# Autodesk Inventor assembly: climber
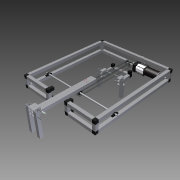
[picture p0: Inventor's stored thumbnail of the model, 180x180]
Saved by Autodesk Inventor 2011 (Build 150239000, 239)
## iProperties
Created: 2013-01-19
Part Number: climber
Document SubType Name: Assembly
Designer: Danny
Author: Danny
## Documents named in this file (18)
- C:\Users\Danny\Documents\GitHub\2013CAD\2013 robot\Spiderbot\climber.iam
- C:\Users\Danny\Documents\GitHub\2013CAD\2013 robot\Spiderbot\28 in 1-16.ipt
- C:\Users\Danny\Documents\GitHub\2013CAD\2013 robot\Spiderbot\24 in 1-16.ipt
- C:\Users\Danny\Documents\GitHub\2013CAD\2013 robot\Spiderbot\2 in 1-16.ipt
- C:\Users\Danny\Documents\GitHub\2013CAD\COTS parts\Plastic_Tubing_Connectors\3-way corner.ipt
- C:\Users\Danny\Documents\GitHub\2013CAD\2013 robot\Spiderbot\cim motor.ipt
- C:\Users\Danny\Documents\GitHub\2013CAD\2013 robot\Spiderbot\cim p80 gearbox.ipt
- C:\Users\Danny\Documents\GitHub\2013CAD\2013 robot\Spiderbot\sprocket.ipt
- C:\Users\Danny\Documents\GitHub\2013CAD\2013 robot\Spiderbot\axle bearing.ipt
- C:\Users\Danny\Documents\GitHub\2013CAD\2013 robot\Spiderbot\30 in 1-2 axle.ipt
- C:\Users\Danny\Documents\GitHub\2013CAD\2013 robot\Spiderbot\climber\Design Accelerator\Key Connection1.iam
- C:\Users\Danny\Documents\GitHub\2013CAD\2013 robot\Spiderbot\chainparts.ipt
- C:\Users\Danny\Documents\GitHub\2013CAD\2013 robot\Spiderbot\screwpin idk man.ipt
- C:\Users\Danny\Documents\GitHub\2013CAD\2013 robot\Spiderbot\short hex bolt.ipt
- C:\Users\Danny\Documents\GitHub\2013CAD\2013 robot\Spiderbot\nylock nut.ipt
- C:\Users\Danny\Documents\GitHub\2013CAD\2013 robot\Spiderbot\longarms.iam
- C:\Users\Danny\Documents\GitHub\2013CAD\2013 robot\Spiderbot\8 in 1-16.ipt
- C:\Users\Danny\Documents\GitHub\2013CAD\2013 robot\Spiderbot\longlongerarms.iam
## Components (55 placed, 17 different names)
1. 28 in 1-16:1 — Mate:26, Flush:57, Flush:58, Flush:59, Flush:60
2. 28 in 1-16:2 — Mate:1, Flush:1, Flush:2, Flush:3, Mate:5, Flush:9, Flush:10, Mate:56, Flush:75
3. 28 in 1-16:3 — Mate:4, Flush:7, Flush:8, Mate:6, Flush:11, Flush:12, Mate:57, Flush:76, Flush:77
4. 28 in 1-16:4 — Mate:25, Flush:53, Flush:54, Flush:55, Flush:56
5. 24 in 1-16:1 — Mate:27, Flush:61, Flush:62, Flush:63, Flush:64, Mate:72, Flush:78, Mate:73
6. 24 in 1-16:2 — Mate:2, Flush:3, Flush:4, Mate:3, Flush:5, Flush:6, Mate:65, Mate:70, Mate:71
7. 2 in 1-16:1 — Mate:14, Flush:27, Flush:28, Mate:19, Flush:37, Flush:38
8. 2 in 1-16:2 — Mate:13, Flush:25, Flush:26, Mate:20, Flush:39, Flush:40
9. 2 in 1-16:3 — Mate:11, Flush:21, Flush:22, Mate:21, Flush:41, Flush:42
10. 2 in 1-16:4 — Mate:12, Flush:23, Flush:24, Mate:22, Flush:43, Flush:44
11. 3-way corner:1 — Mate:5, Flush:9, Flush:10, Mate:14, Flush:27, Flush:28, Mate:79, Flush:82, Flush:83
12. 3-way corner:2 — Mate:1, Flush:1, Flush:2, Mate:2, Flush:4, Mate:15, Flush:29, Flush:30
13. 3-way corner:3 — Mate:11, Flush:21, Flush:22, Flush:84
14. 3-way corner:4 — Mate:12, Flush:23, Flush:24, Mate:82, Flush:89, Flush:91
15. 3-way corner:5 — Mate:19, Flush:37, Flush:38, Mate:26, Flush:57, Flush:58, Mate:77, Flush:80, Flush:81
16. 3-way corner:6 — Mate:18, Flush:35, Flush:36, Flush:55, Flush:56, Flush:63, Flush:64
17. 3-way corner:7 — Mate:22, Flush:43, Flush:44, Mate:80, Flush:85, Flush:86
18. 3-way corner:8 — Mate:6, Flush:11, Flush:12, Mate:13, Flush:25, Flush:26, Flush:90
19. 3-way corner:9 — Mate:3, Flush:5, Flush:6, Mate:4, Flush:7, Flush:8, Mate:16, Flush:31, Flush:32
20. 3-way corner:10 — Mate:17, Flush:33, Flush:34, Flush:59, Flush:60, Mate:27, Flush:61, Flush:62
21. 2 in 1-16:5 — Mate:15, Flush:29, Flush:30, Mate:17, Flush:33, Flush:34
22. 2 in 1-16:6 — Mate:16, Flush:31, Flush:32, Mate:18, Flush:35, Flush:36
23. 3-way corner:11 — Mate:20, Flush:39, Flush:40, Mate:25, Flush:53, Flush:54, Mate:81, Flush:87, Flush:88
24. 3-way corner:12 — Mate:21, Flush:41, Flush:42, Mate:78
25. cim motor:1 — Mate:48
26. cim p80 gearbox:1 — Mate:32, Mate:34, Flush:69, Mate:48, Mate:65
27. sprocket:2 — Mate:32, Flush:69, Mate:67
28. sprocket:3 — Mate:34, Mate:69
29. Key Connection:1 [sub-assembly] — Mate:63, Mate:64
30. 30 in 1-2 axle:2 — Mate:58, Mate:59, Flush:77, Mate:60, Mate:61, Mate:62, Mate:63, Mate:64
31. axle bearing:3 — Mate:57, Flush:76, Mate:59
32. axle bearing:4 — Mate:56, Flush:75, Mate:58
33. sprocket:7 — Mate:60, Mate:68
34. sprocket:8 — Mate:61, Mate:62, Mate:66
35. chainparts:1 — Mate:68, Mate:69, Mate:88, Mate:89
36. chainparts:2 — Mate:66, Mate:67, Mate:76, Flush:79, Mate:87, Mate:90, Mate:91
37. screwpin idk man:1
38. screwpin idk man:2 — Mate:70, Mate:71
39. 2 in 1-16:7 — Mate:72, Flush:78, Mate:75
40. Chassis_HexBolt_375x16x7_AndyMark_am-1055:2 — Mate:73, Mate:74
41. nylock nut:1 — Mate:74, Mate:75
42. longarms:1 [sub-assembly] — Mate:76, Flush:79, Mate:83, Mate:84, Mate:85, Mate:86
43. 8 in 1-16:1 — Mate:80, Flush:85, Flush:86, Mate:81, Flush:87, Flush:88
44. 8 in 1-16:2 — Mate:79, Flush:82, Flush:83, Flush:84
45. 8 in 1-16:3 — Mate:77, Flush:80, Flush:81, Mate:78
46. 8 in 1-16:4 — Mate:82, Flush:89, Flush:90, Flush:91
47. screwpin idk man:3 — Mate:83
48. screwpin idk man:4 — Mate:84
49. screwpin idk man:5 — Mate:85
50. screwpin idk man:6 — Mate:86
51. longlongerarms:1 [sub-assembly] — Mate:87
52. screwpin idk man:7 — Mate:89
53. screwpin idk man:8 — Mate:91
54. screwpin idk man:9 — Mate:88
55. screwpin idk man:10 — Mate:90
## Relationships (126: Flush 66, Mate 60)
- Mate:1: 28 in 1-16:2 ↔ 3-way corner:2
- Flush:1: 28 in 1-16:2 ↔ 3-way corner:2
- Flush:2: 28 in 1-16:2 ↔ 3-way corner:2
- Mate:2: 24 in 1-16:2 ↔ 3-way corner:2
- Flush:3: 28 in 1-16:2 ↔ 24 in 1-16:2
- Flush:4: 24 in 1-16:2 ↔ 3-way corner:2
- Mate:3: 24 in 1-16:2 ↔ 3-way corner:9
- Flush:5: 24 in 1-16:2 ↔ 3-way corner:9
- Flush:6: 24 in 1-16:2 ↔ 3-way corner:9
- Mate:4: 28 in 1-16:3 ↔ 3-way corner:9
- Flush:7: 28 in 1-16:3 ↔ 3-way corner:9
- Flush:8: 28 in 1-16:3 ↔ 3-way corner:9
- Mate:5: 28 in 1-16:2 ↔ 3-way corner:1
- Flush:9: 28 in 1-16:2 ↔ 3-way corner:1
- Flush:10: 28 in 1-16:2 ↔ 3-way corner:1
- Mate:6: 28 in 1-16:3 ↔ 3-way corner:8
- Flush:11: 28 in 1-16:3 ↔ 3-way corner:8
- Flush:12: 28 in 1-16:3 ↔ 3-way corner:8
- Mate:11: 2 in 1-16:3 ↔ 3-way corner:3
- Flush:21: 2 in 1-16:3 ↔ 3-way corner:3
- Flush:22: 2 in 1-16:3 ↔ 3-way corner:3
- Mate:12: 2 in 1-16:4 ↔ 3-way corner:4
- Flush:23: 2 in 1-16:4 ↔ 3-way corner:4
- Flush:24: 2 in 1-16:4 ↔ 3-way corner:4
- Mate:13: 2 in 1-16:2 ↔ 3-way corner:8
- Flush:25: 2 in 1-16:2 ↔ 3-way corner:8
- Flush:26: 2 in 1-16:2 ↔ 3-way corner:8
- Mate:14: 2 in 1-16:1 ↔ 3-way corner:1
- Flush:27: 2 in 1-16:1 ↔ 3-way corner:1
- Flush:28: 2 in 1-16:1 ↔ 3-way corner:1
- Mate:15: 3-way corner:2 ↔ 2 in 1-16:5
- Flush:29: 3-way corner:2 ↔ 2 in 1-16:5
- Flush:30: 3-way corner:2 ↔ 2 in 1-16:5
- Mate:16: 3-way corner:9 ↔ 2 in 1-16:6
- Flush:31: 3-way corner:9 ↔ 2 in 1-16:6
- Flush:32: 3-way corner:9 ↔ 2 in 1-16:6
- Mate:17: 3-way corner:10 ↔ 2 in 1-16:5
- Flush:33: 3-way corner:10 ↔ 2 in 1-16:5
- Flush:34: 3-way corner:10 ↔ 2 in 1-16:5
- Mate:18: 3-way corner:6 ↔ 2 in 1-16:6
- Flush:35: 3-way corner:6 ↔ 2 in 1-16:6
- Flush:36: 3-way corner:6 ↔ 2 in 1-16:6
- Mate:19: 2 in 1-16:1 ↔ 3-way corner:5
- Flush:37: 2 in 1-16:1 ↔ 3-way corner:5
- Flush:38: 2 in 1-16:1 ↔ 3-way corner:5
- Mate:20: 2 in 1-16:2 ↔ 3-way corner:11
- Flush:39: 2 in 1-16:2 ↔ 3-way corner:11
- Flush:40: 2 in 1-16:2 ↔ 3-way corner:11
- Mate:21: 2 in 1-16:3 ↔ 3-way corner:12
- Flush:41: 2 in 1-16:3 ↔ 3-way corner:12
- Flush:42: 2 in 1-16:3 ↔ 3-way corner:12
- Mate:22: 2 in 1-16:4 ↔ 3-way corner:7
- Flush:43: 2 in 1-16:4 ↔ 3-way corner:7
- Flush:44: 2 in 1-16:4 ↔ 3-way corner:7
- Mate:25: 28 in 1-16:4 ↔ 3-way corner:11
- Flush:53: 28 in 1-16:4 ↔ 3-way corner:11
- Flush:54: 28 in 1-16:4 ↔ 3-way corner:11
- Flush:55: 28 in 1-16:4 ↔ 3-way corner:6
- Flush:56: 28 in 1-16:4 ↔ 3-way corner:6
- Mate:26: 28 in 1-16:1 ↔ 3-way corner:5
- Flush:57: 28 in 1-16:1 ↔ 3-way corner:5
- Flush:58: 28 in 1-16:1 ↔ 3-way corner:5
- Flush:59: 28 in 1-16:1 ↔ 3-way corner:10
- Flush:60: 28 in 1-16:1 ↔ 3-way corner:10
- Mate:27: 24 in 1-16:1 ↔ 3-way corner:10
- Flush:61: 24 in 1-16:1 ↔ 3-way corner:10
- Flush:62: 24 in 1-16:1 ↔ 3-way corner:10
- Flush:63: 24 in 1-16:1 ↔ 3-way corner:6
- Flush:64: 24 in 1-16:1 ↔ 3-way corner:6
- Mate:32: cim p80 gearbox:1 ↔ sprocket:2
- Mate:34: cim p80 gearbox:1 ↔ sprocket:3
- Flush:69: cim p80 gearbox:1 ↔ sprocket:2
- Mate:48: cim motor:1 ↔ cim p80 gearbox:1
- Mate:56: 28 in 1-16:2 ↔ axle bearing:4
- Flush:75: 28 in 1-16:2 ↔ axle bearing:4
- Mate:57: 28 in 1-16:3 ↔ axle bearing:3
- Flush:76: 28 in 1-16:3 ↔ axle bearing:3
- Mate:58: 30 in 1-2 axle:2 ↔ axle bearing:4
- Mate:59: 30 in 1-2 axle:2 ↔ axle bearing:3
- Flush:77: 28 in 1-16:3 ↔ 30 in 1-2 axle:2
- Mate:60: 30 in 1-2 axle:2 ↔ sprocket:7
- Mate:61: 30 in 1-2 axle:2 ↔ sprocket:8
- Mate:62: 30 in 1-2 axle:2 ↔ sprocket:8
- Mate:63: Key Connection:1 ↔ 30 in 1-2 axle:2
- Mate:64: Key Connection:1 ↔ 30 in 1-2 axle:2
- Mate:65: 24 in 1-16:2 ↔ cim p80 gearbox:1
- Mate:66: sprocket:8 ↔ chainparts:2
- Mate:67: sprocket:2 ↔ chainparts:2
- Mate:68: sprocket:7 ↔ chainparts:1
- Mate:69: sprocket:3 ↔ chainparts:1
- Mate:70: 24 in 1-16:2 ↔ screwpin idk man:2
- Mate:71: 24 in 1-16:2 ↔ screwpin idk man:2
- Mate:72: 24 in 1-16:1 ↔ 2 in 1-16:7
- Flush:78: 24 in 1-16:1 ↔ 2 in 1-16:7
- Mate:73: 24 in 1-16:1 ↔ Chassis_HexBolt_375x16x7_AndyMark_am-1055:2
- Mate:74: Chassis_HexBolt_375x16x7_AndyMark_am-1055:2 ↔ nylock nut:1
- Mate:75: 2 in 1-16:7 ↔ nylock nut:1
- Mate:76: chainparts:2 ↔ longarms:1
- Flush:79: chainparts:2 ↔ longarms:1
- Mate:77: 3-way corner:5 ↔ 8 in 1-16:3
- Flush:80: 3-way corner:5 ↔ 8 in 1-16:3
- Flush:81: 3-way corner:5 ↔ 8 in 1-16:3
- Mate:78: 3-way corner:12 ↔ 8 in 1-16:3
- Mate:79: 3-way corner:1 ↔ 8 in 1-16:2
- Flush:82: 3-way corner:1 ↔ 8 in 1-16:2
- Flush:83: 3-way corner:1 ↔ 8 in 1-16:2
- Flush:84: 3-way corner:3 ↔ 8 in 1-16:2
- Mate:80: 3-way corner:7 ↔ 8 in 1-16:1
- Flush:85: 3-way corner:7 ↔ 8 in 1-16:1
- Flush:86: 3-way corner:7 ↔ 8 in 1-16:1
- Mate:81: 3-way corner:11 ↔ 8 in 1-16:1
- Flush:87: 3-way corner:11 ↔ 8 in 1-16:1
- Flush:88: 3-way corner:11 ↔ 8 in 1-16:1
- Mate:82: 3-way corner:4 ↔ 8 in 1-16:4
- Flush:89: 3-way corner:4 ↔ 8 in 1-16:4
- Flush:90: 3-way corner:8 ↔ 8 in 1-16:4
- Flush:91: 3-way corner:4 ↔ 8 in 1-16:4
- Mate:83: longarms:1 ↔ screwpin idk man:3
- Mate:84: longarms:1 ↔ screwpin idk man:4
- Mate:85: longarms:1 ↔ screwpin idk man:5
- Mate:86: longarms:1 ↔ screwpin idk man:6
- Mate:87: chainparts:2 ↔ longlongerarms:1
- Mate:88: chainparts:1 ↔ screwpin idk man:9
- Mate:89: chainparts:1 ↔ screwpin idk man:7
- Mate:90: chainparts:2 ↔ screwpin idk man:10
- Mate:91: chainparts:2 ↔ screwpin idk man:8
